# Autodesk Inventor assembly: 543979 DGSL-12-50-Y3A---(0)
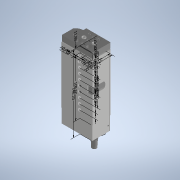
[picture p0: Inventor's stored thumbnail of the model, 180x180]
Saved by Autodesk Inventor 2021 (Build 250183000, 183)
## iProperties
Category: PARTsolutions
Company: FESTO
Created: 2026-04-25
Part Number: 543979 DGSL-12-50-Y3A---(0)
Catalog Web Link: www.3dfindit.com
Description: DGSL-mini slide
Vendor: FESTO
Document SubType Name: Assembly
Designer: psAdmin
Manufacturer: FESTO
Mass: 855 g
Surface Area: 767.952 cm^2
Volume: 230.478 cm^3
Density: 3.70968 g/cm^3
Title: 543979 DGSL-12-50-Y3A
Author: Cadenas PARTsolutions
Comments: mini slide
PSOL_IDENT_0: {ATYP=ASSISTANT},{DATA=script=$CADENAS_DATA/23d-libs/festo/webfesto.vbb&M_FAMILY=DGSL&M_GROUP=01&M_P
PSOL_IDENT_1: ARTNO=543979&IDCODE1=DGSL-12-50-Y3A&IDCODE2=&customer_number_cns=&MATES=1&LOD=HI&LOCKERP=0&SINGLEPAR
PSOL_IDENT_2: T=1}
NB: 543979 DGSL-12-50-Y3A---(0)
NN: DGSL
NT: mini slide
NBSYN: $TNR. $TYP.---($HUBST.)
LINA: 543979 DGSL-12-50-Y3A
CATALOG: Festo
TNR: 543979
TYP: DGSL-12-50-Y3A
HUBST: 0
CNSMASSEXACT: 0.855
GTIN: 4052568005887
SUPPLIER: FESTO
ARTICLENO: 543979 DGSL-12-50-Y3A---(0)
BOMINFO: 543979 DGSL-12-50-Y3A
CREATOR: CADENAS GmbH
## Documents named in this file (7)
- e:\temp\worker_COMMON_260\temp\tmp_3564_2_dLXvV\format_0\543979 DGSL-12-50-Y3A---(0).iam
- e:\temp\worker_COMMON_260\temp\tmp_3564_2_dLXvV\format_0\DGSL-12---(50-0-0-30-zr).ipt
- e:\temp\worker_COMMON_260\temp\tmp_3564_2_dLXvV\format_0\548072 DYSW-7-10-Y1F---(SD_0).ipt
- e:\temp\worker_COMMON_260\temp\tmp_3564_2_dLXvV\format_0\174308 B-M5-B.ipt
- e:\temp\worker_COMMON_260\temp\tmp_3564_2_dLXvV\format_0\686786 DGSL-12-AS.ipt
- e:\temp\worker_COMMON_260\temp\tmp_3564_2_dLXvV\format_0\DGSL-12---(50-0-JP).ipt
- e:\temp\worker_COMMON_260\temp\tmp_3564_2_dLXvV\format_0\8210495 ZBH-7.ipt
## Components (13 placed, 6 different names)
1. DGSL-12---(50-0-0-30-zr):1 — IP_SD_XY@1 <-> IP_DGSL_XY@2, IP_SD_Z@1 <-> IP_DGSL_Z@2, IP_SD_YZ@1 <-> IP_DGSL_YZ@2, IP_BS_1_XY@1 <-> ANBAU_XY@3, IP_BS_1_Z@1 <-> ANBAU_Z@3, IP_BS_1_YZ@1 <-> ANBAU_YZ@3, IP_BS_2_XY@1 <-> ANBAU_XY@4, IP_BS_2_Z@1 <-> ANBAU_Z@4, IP_BS_2_YZ@1 <-> ANBAU_YZ@4, IP_A1_XY@1 <-> ANBAU_XY@5, IP_A1_Z@1 <-> ANBAU_Z@5, IP_A1_YZ@1 <-> ANBAU_YZ@5, IP_KS_XY@1 <-> ANBAU_XY@6, IP_KS_Z@1 <-> ANBAU_Z@6, IP_KS_YZ@1 <-> ANBAU_YZ@6
2. 548072 DYSW-7-10-Y1F---(SD_0):1 — IP_SD_XY@1 <-> IP_DGSL_XY@2, IP_SD_Z@1 <-> IP_DGSL_Z@2, IP_SD_YZ@1 <-> IP_DGSL_YZ@2
3. 174308 B-M5-B:1 — IP_BS_1_XY@1 <-> ANBAU_XY@3, IP_BS_1_Z@1 <-> ANBAU_Z@3, IP_BS_1_YZ@1 <-> ANBAU_YZ@3
4. 174308 B-M5-B:2 — IP_BS_2_XY@1 <-> ANBAU_XY@4, IP_BS_2_Z@1 <-> ANBAU_Z@4, IP_BS_2_YZ@1 <-> ANBAU_YZ@4
5. 686786 DGSL-12-AS:1 — IP_A1_XY@1 <-> ANBAU_XY@5, IP_A1_Z@1 <-> ANBAU_Z@5, IP_A1_YZ@1 <-> ANBAU_YZ@5
6. DGSL-12---(50-0-JP):1 — IP_KS_XY@1 <-> ANBAU_XY@6, IP_KS_Z@1 <-> ANBAU_Z@6, IP_KS_YZ@1 <-> ANBAU_YZ@6, IP_SD_XY@6 <-> IP_DGSL_XY@7, IP_SD_Z@6 <-> IP_DGSL_Z@7, IP_SD_YZ@6 <-> IP_DGSL_YZ@7, CSL_2_1_XY@6 <-> ANBAU_XY@8, CSL_2_1_Z@6 <-> ANBAU_Z@8, CSL_2_1_YZ@6 <-> ANBAU_YZ@8, CSL_2_2_XY@6 <-> ANBAU_XY@9, CSL_2_2_Z@6 <-> ANBAU_Z@9, CSL_2_2_YZ@6 <-> ANBAU_YZ@9, CSL_3_1_XY@6 <-> ANBAU_XY@10, CSL_3_1_Z@6 <-> ANBAU_Z@10, CSL_3_1_YZ@6 <-> ANBAU_YZ@10, CSL_3_2_XY@6 <-> ANBAU_XY@11, CSL_3_2_Z@6 <-> ANBAU_Z@11, CSL_3_2_YZ@6 <-> ANBAU_YZ@11
7. 548072 DYSW-7-10-Y1F---(SD_0):2 — IP_SD_XY@6 <-> IP_DGSL_XY@7, IP_SD_Z@6 <-> IP_DGSL_Z@7, IP_SD_YZ@6 <-> IP_DGSL_YZ@7
8. 8210495 ZBH-7:1 — CSL_2_1_XY@6 <-> ANBAU_XY@8, CSL_2_1_Z@6 <-> ANBAU_Z@8, CSL_2_1_YZ@6 <-> ANBAU_YZ@8
9. 8210495 ZBH-7:2 — CSL_2_2_XY@6 <-> ANBAU_XY@9, CSL_2_2_Z@6 <-> ANBAU_Z@9, CSL_2_2_YZ@6 <-> ANBAU_YZ@9
10. 8210495 ZBH-7:3 — CSL_3_1_XY@6 <-> ANBAU_XY@10, CSL_3_1_Z@6 <-> ANBAU_Z@10, CSL_3_1_YZ@6 <-> ANBAU_YZ@10
11. 8210495 ZBH-7:4 — CSL_3_2_XY@6 <-> ANBAU_XY@11, CSL_3_2_Z@6 <-> ANBAU_Z@11, CSL_3_2_YZ@6 <-> ANBAU_YZ@11
12. 8210495 ZBH-7:5
13. 8210495 ZBH-7:6
## Relationships (30: Mate 18, Angle 10, Flush 2)
- IP_SD_XY@1 <-> IP_DGSL_XY@2 [Flush] (36.45 mm): DGSL-12---(50-0-0-30-zr):1 ↔ 548072 DYSW-7-10-Y1F---(SD_0):1
- IP_SD_Z@1 <-> IP_DGSL_Z@2 [Mate]: DGSL-12---(50-0-0-30-zr):1 ↔ 548072 DYSW-7-10-Y1F---(SD_0):1
- IP_SD_YZ@1 <-> IP_DGSL_YZ@2 [Angle] (0 deg): DGSL-12---(50-0-0-30-zr):1 ↔ 548072 DYSW-7-10-Y1F---(SD_0):1
- IP_BS_1_XY@1 <-> ANBAU_XY@3 [Mate]: DGSL-12---(50-0-0-30-zr):1 ↔ 174308 B-M5-B:1
- IP_BS_1_Z@1 <-> ANBAU_Z@3 [Mate]: DGSL-12---(50-0-0-30-zr):1 ↔ 174308 B-M5-B:1
- IP_BS_1_YZ@1 <-> ANBAU_YZ@3 [Angle] (0 deg): DGSL-12---(50-0-0-30-zr):1 ↔ 174308 B-M5-B:1
- IP_BS_2_XY@1 <-> ANBAU_XY@4 [Mate]: DGSL-12---(50-0-0-30-zr):1 ↔ 174308 B-M5-B:2
- IP_BS_2_Z@1 <-> ANBAU_Z@4 [Mate]: DGSL-12---(50-0-0-30-zr):1 ↔ 174308 B-M5-B:2
- IP_BS_2_YZ@1 <-> ANBAU_YZ@4 [Angle] (0 deg): DGSL-12---(50-0-0-30-zr):1 ↔ 174308 B-M5-B:2
- IP_A1_XY@1 <-> ANBAU_XY@5 [Mate]: DGSL-12---(50-0-0-30-zr):1 ↔ 686786 DGSL-12-AS:1
- IP_A1_Z@1 <-> ANBAU_Z@5 [Mate]: DGSL-12---(50-0-0-30-zr):1 ↔ 686786 DGSL-12-AS:1
- IP_A1_YZ@1 <-> ANBAU_YZ@5 [Angle] (0 deg): DGSL-12---(50-0-0-30-zr):1 ↔ 686786 DGSL-12-AS:1
- IP_KS_XY@1 <-> ANBAU_XY@6 [Mate]: DGSL-12---(50-0-0-30-zr):1 ↔ DGSL-12---(50-0-JP):1
- IP_KS_Z@1 <-> ANBAU_Z@6 [Mate]: DGSL-12---(50-0-0-30-zr):1 ↔ DGSL-12---(50-0-JP):1
- IP_KS_YZ@1 <-> ANBAU_YZ@6 [Angle] (0 deg): DGSL-12---(50-0-0-30-zr):1 ↔ DGSL-12---(50-0-JP):1
- IP_SD_XY@6 <-> IP_DGSL_XY@7 [Flush] (38.55 mm): DGSL-12---(50-0-JP):1 ↔ 548072 DYSW-7-10-Y1F---(SD_0):2
- IP_SD_Z@6 <-> IP_DGSL_Z@7 [Mate]: DGSL-12---(50-0-JP):1 ↔ 548072 DYSW-7-10-Y1F---(SD_0):2
- IP_SD_YZ@6 <-> IP_DGSL_YZ@7 [Angle] (0 deg): DGSL-12---(50-0-JP):1 ↔ 548072 DYSW-7-10-Y1F---(SD_0):2
- CSL_2_1_XY@6 <-> ANBAU_XY@8 [Mate] (1.6 mm): DGSL-12---(50-0-JP):1 ↔ 8210495 ZBH-7:1
- CSL_2_1_Z@6 <-> ANBAU_Z@8 [Mate]: DGSL-12---(50-0-JP):1 ↔ 8210495 ZBH-7:1
- CSL_2_1_YZ@6 <-> ANBAU_YZ@8 [Angle] (0 deg): DGSL-12---(50-0-JP):1 ↔ 8210495 ZBH-7:1
- CSL_2_2_XY@6 <-> ANBAU_XY@9 [Mate] (1.6 mm): DGSL-12---(50-0-JP):1 ↔ 8210495 ZBH-7:2
- CSL_2_2_Z@6 <-> ANBAU_Z@9 [Mate]: DGSL-12---(50-0-JP):1 ↔ 8210495 ZBH-7:2
- CSL_2_2_YZ@6 <-> ANBAU_YZ@9 [Angle] (0 deg): DGSL-12---(50-0-JP):1 ↔ 8210495 ZBH-7:2
- CSL_3_1_XY@6 <-> ANBAU_XY@10 [Mate] (1.6 mm): DGSL-12---(50-0-JP):1 ↔ 8210495 ZBH-7:3
- CSL_3_1_Z@6 <-> ANBAU_Z@10 [Mate]: DGSL-12---(50-0-JP):1 ↔ 8210495 ZBH-7:3
- CSL_3_1_YZ@6 <-> ANBAU_YZ@10 [Angle] (0 deg): DGSL-12---(50-0-JP):1 ↔ 8210495 ZBH-7:3
- CSL_3_2_XY@6 <-> ANBAU_XY@11 [Mate] (1.6 mm): DGSL-12---(50-0-JP):1 ↔ 8210495 ZBH-7:4
- CSL_3_2_Z@6 <-> ANBAU_Z@11 [Mate]: DGSL-12---(50-0-JP):1 ↔ 8210495 ZBH-7:4
- CSL_3_2_YZ@6 <-> ANBAU_YZ@11 [Angle] (0 deg): DGSL-12---(50-0-JP):1 ↔ 8210495 ZBH-7:4
